# Autodesk Inventor assembly: Vex Wheel Assembly
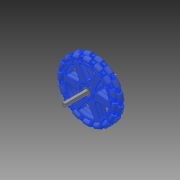
[picture p0: Inventor's stored thumbnail of the model, 180x180]
Saved by Autodesk Inventor 2013 (Build 170138000, 138)
## iProperties
Created: 2013-01-10
Part Number: Vex Wheel Assembly
Document SubType Name: Assembly
Designer: Naphat
Author: Naphat
## Documents named in this file (5)
- C:\Users\carneeki\Desktop\Kiwi Robot\Vex Wheel\Vex Wheel Assembly.iam
- C:\Users\carneeki\Desktop\Kiwi Robot\Imported Components\217-2613.20121203\217-2613.20121203.iam
- C:\Users\carneeki\Desktop\Kiwi Robot\217-2592.20121203.ipt
- C:\Users\carneeki\Desktop\Kiwi Robot\Hex Shaft.ipt
- C:\Users\carneeki\Desktop\Kiwi Robot\Vex Wheel\ShaftCollar.ipt
## Components (5 placed, 4 different names)
1. 217-2613.20121203:1 [sub-assembly] — Insert:2, Insert:3
2. 217-2592.20121203:1 — Mate:1, Insert:2, Mate:2
3. Hex Shaft:1 — Insert:1
4. ShaftCollar:1 — Insert:1, Mate:1
5. ShaftCollar:2 — Mate:2, Insert:3
## Relationships (5: Insert 3, Mate 2)
- Insert:1 (56 mm): Hex Shaft:1 ↔ ShaftCollar:1
- Mate:1: 217-2592.20121203:1 ↔ ShaftCollar:1
- Insert:2: 217-2613.20121203:1 ↔ 217-2592.20121203:1
- Mate:2: 217-2592.20121203:1 ↔ ShaftCollar:2
- Insert:3: 217-2613.20121203:1 ↔ ShaftCollar:2
